# Autodesk Inventor assembly: strut
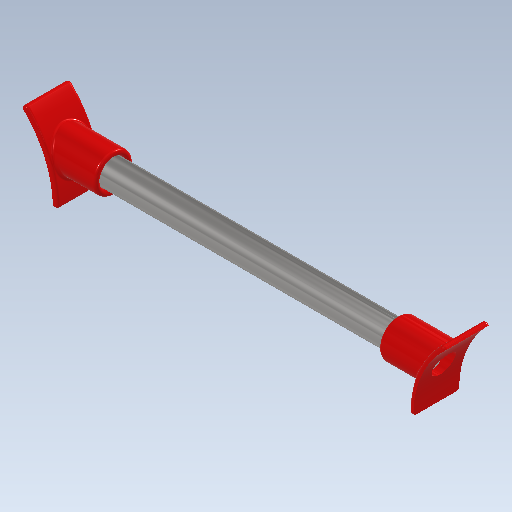
[picture p0: Inventor's stored thumbnail of the model, 512x512]
Saved by Autodesk Inventor 2020.2 (Build 242310000, 310)
## iProperties
Created: 2020-03-22
Part Number: strut
Document SubType Name: Assembly
Designer: agmle
Mass: 560.594 g
Surface Area: 1083.17 cm^2
Volume: 159.493 cm^3
Density: 3.51486 g/cm^3
Author: agmle
## Documents named in this file (3)
- M:\documents\Inventor\AutoBuoy\hull\strut.iam
- M:\documents\Inventor\AutoBuoy\hull\strut.ipt
- M:\documents\Inventor\AutoBuoy\hull\strut_flange.ipt
## Components (3 placed, 2 different names)
1. strut:1 — Insert:1, Insert:2
2. strut_flange:1 — Insert:1, Flush:1, Mate:1, Mate:2
3. strut_flange:2 — Insert:2, Flush:1
## Relationships (5: Insert 2, Mate 2, Flush 1)
- Insert:1: strut:1 ↔ strut_flange:1
- Insert:2: strut:1 ↔ strut_flange:2
- Flush:1: strut_flange:1 ↔ strut_flange:2
- Mate:1: strut_flange:1
- Mate:2: strut_flange:1
